# Autodesk Inventor assembly: Elevatorcarv2
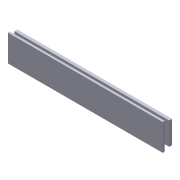
[picture p0: Inventor's stored thumbnail of the model, 180x180]
Saved by Autodesk Inventor 2015 (Build 190159000, 159)
## iProperties
Created: 2015-01-19
Part Number: Elevatorcarv2
Document SubType Name: Assembly
Designer: Tanner
Author: Tanner
## Documents named in this file (4)
- C:\Users\Tanner\Documents\Inventor\ElevatorCAD\Elevatorcarv2.iam
- C:\Users\Tanner\Documents\Inventor\ElevatorCAD\Elevatorcarv2bottom.ipt
- C:\Users\Tanner\Documents\Inventor\ElevatorCAD\BallBearing.ipt
- C:\Users\Tanner\Documents\Inventor\ElevatorCAD\Elevatorcarv2top.ipt
## Components (6 placed, 3 different names)
1. BallBearing:1 — Mate:1, Tangent:2, Tangent:7, Mate:5
2. BallBearing:2 — Mate:2, Tangent:1, Tangent:6, Tangent:7
3. BallBearing:3 — Mate:4, Tangent:3, Tangent:8
4. BallBearing:4 — Mate:3, Tangent:4, Tangent:5, Tangent:8
5. Elevatorcarv2bottom:1 — Mate:1, Mate:2, Mate:3, Mate:4, Tangent:1, Tangent:2, Tangent:3, Tangent:4, Tangent:5, Tangent:6, Flush:2, Flush:3
6. Elevatorcarv2top:1 — Mate:5, Flush:2, Flush:3
## Relationships (15: Tangent 8, Mate 5, Flush 2)
- Mate:1: BallBearing:1 ↔ Elevatorcarv2bottom:1
- Mate:2: BallBearing:2 ↔ Elevatorcarv2bottom:1
- Mate:3: BallBearing:4 ↔ Elevatorcarv2bottom:1
- Mate:4: BallBearing:3 ↔ Elevatorcarv2bottom:1
- Tangent:1 (6.8326 mm): BallBearing:2 ↔ Elevatorcarv2bottom:1
- Tangent:2 (6.8326 mm): BallBearing:1 ↔ Elevatorcarv2bottom:1
- Tangent:3 (6.8326 mm): BallBearing:3 ↔ Elevatorcarv2bottom:1
- Tangent:4 (6.8326 mm): BallBearing:4 ↔ Elevatorcarv2bottom:1
- Tangent:5 (14.4526 mm): BallBearing:4 ↔ Elevatorcarv2bottom:1
- Tangent:6 (14.4526 mm): BallBearing:2 ↔ Elevatorcarv2bottom:1
- Tangent:7 (16.2052 mm): BallBearing:1 ↔ BallBearing:2
- Tangent:8 (16.2052 mm): BallBearing:3 ↔ BallBearing:4
- Mate:5: BallBearing:1 ↔ Elevatorcarv2top:1
- Flush:2: Elevatorcarv2bottom:1 ↔ Elevatorcarv2top:1
- Flush:3 (-3.0353 mm): Elevatorcarv2bottom:1 ↔ Elevatorcarv2top:1
## Named parameters: noah = 6.8326 mm, tanner = 14.4526 mm, stupid = 16.2052 mm
